# Autodesk Inventor assembly: Fixture Assembly
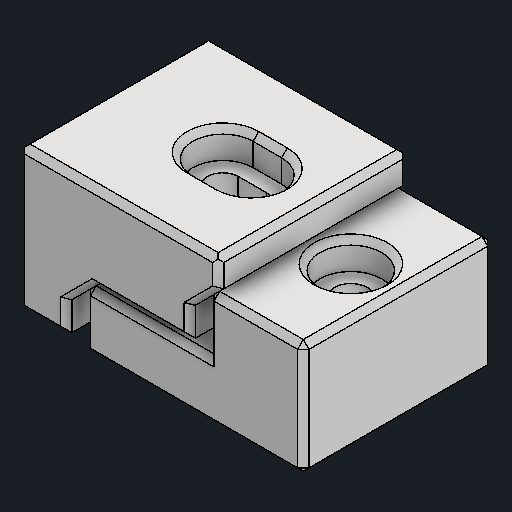
[picture p0: Inventor's stored thumbnail of the model, 512x512]
Saved by Autodesk Inventor 2026.2 (Build 302298000, 298)
## iProperties
Created: 2026-07-19
Part Number: Fixture Assembly
Document SubType Name: Assembly
Designer: JoshuaEah
Author: JoshuaEah
## Documents named in this file (3)
- C:\Users\JoshuaEah\Documents\GitHub\Designed-Trinkets\Guitar\Modular Pedalboard\Fixtures\M3 Version\Fixture Assembly (M3).iam
- C:\Users\JoshuaEah\Documents\GitHub\Designed-Trinkets\Guitar\Modular Pedalboard\Fixtures\M3 Version\Moving Jaw (M3).ipt
- C:\Users\JoshuaEah\Documents\GitHub\Designed-Trinkets\Guitar\Modular Pedalboard\Fixtures\M3 Version\Fixed Jaw (M3).ipt
## Components (2 placed, 2 different names)
1. Moving Jaw (M3):1 — Flush:1, Transitional:2, Angle:1
2. Fixed Jaw (M3):1 — Flush:1, Transitional:2, Angle:1
## Relationships (3: Flush 1, Transitional 1, Angle 1)
- Flush:1: Moving Jaw (M3):1 ↔ Fixed Jaw (M3):1
- Transitional:2: Moving Jaw (M3):1 ↔ Fixed Jaw (M3):1
- Angle:1 (90 deg): Moving Jaw (M3):1 ↔ Fixed Jaw (M3):1
